# Autodesk Inventor assembly: Raspberry Pi 3
(part 2 of 2)
276. Raspberry Pi 3319_276
277. Raspberry Pi 3320_277
278. Raspberry Pi 3321_278
279. Raspberry Pi 3322_279
280. Raspberry Pi 3323_280
281. Raspberry Pi 3324_281
282. Raspberry Pi 3325_282
283. Raspberry Pi 3326_283
284. Raspberry Pi 3327_284
285. Raspberry Pi 3328_285
286. Raspberry Pi 3329_286
287. Raspberry Pi 3330_287
288. Raspberry Pi 3331_288
289. Raspberry Pi 3332_289
290. Raspberry Pi 3333_290
291. Raspberry Pi 3334_291
292. Raspberry Pi 3335_292
293. Raspberry Pi 3336_293
294. Raspberry Pi 3337_294
295. Raspberry Pi 3338_295
296. Raspberry Pi 3339_296
297. Raspberry Pi 3340_297
298. Raspberry Pi 3341_298
299. Raspberry Pi 3342_299
300. Raspberry Pi 3343_300
301. Raspberry Pi 3344_301
302. Raspberry Pi 3345_302
303. Raspberry Pi 3346_303
304. Raspberry Pi 3347_304
305. Raspberry Pi 3348_305
306. Raspberry Pi 3349_306
307. Raspberry Pi 3350_307
308. Raspberry Pi 3351_308
309. Raspberry Pi 3352_309
310. Raspberry Pi 3353_310
311. Raspberry Pi 3354_311
312. Raspberry Pi 327_312
313. Raspberry Pi 340_313
314. Raspberry Pi 344_314
315. Raspberry Pi 344_315
316. Raspberry Pi 340_316
317. Raspberry Pi 344_317
318. Raspberry Pi 340_318
319. Raspberry Pi 344_319
320. Raspberry Pi 340_320
321. Raspberry Pi 344_321
322. Raspberry Pi 340_322
323. Raspberry Pi 340_323
324. Raspberry Pi 344_324
325. Raspberry Pi 340_325
326. Raspberry Pi 344_326
327. Raspberry Pi 3357_327
328. Raspberry Pi 3355_328
329. Raspberry Pi 3356_329
330. Raspberry Pi 374_330
331. Raspberry Pi 3141_331
332. Raspberry Pi 374_332
333. Raspberry Pi 374_333
334. Raspberry Pi 374_334
335. Part2^Raspberry Pi 3_335
336. Raspberry Pi 3360_336
337. Part4^Raspberry Pi 3_337
338. Raspberry Pi 3159_338
339. Raspberry Pi 3158_339
340. Raspberry Pi 3160_340
341. Raspberry Pi 3162_341
342. Raspberry Pi 3161_342
343. Raspberry Pi 359_343
344. Raspberry Pi 3165_344
345. Raspberry Pi 353_345
346. Raspberry Pi 3164_346
347. Raspberry Pi 3163_347
348. Raspberry Pi 355_348
349. Raspberry Pi 3168_349
350. Raspberry Pi 3170_350
351. Raspberry Pi 3169_351
352. Raspberry Pi 3171_352
353. Raspberry Pi 3167_353
354. Raspberry Pi 3166_354
355. Raspberry Pi 353_355
356. Raspberry Pi 3165_356
357. Raspberry Pi 3163_357
358. Raspberry Pi 3164_358
359. Solder2_359
360. Solder2_360
361. Solder2_361
362. Solder2_362
363. Solder2_363
364. Solder2_364
365. Solder2_365
366. Solder2_366
367. Solder2_367
368. Solder2_368
369. Solder2_369
370. Raspberry Pi 3359_370
371. Solder2_371
372. Solder2_372
373. Solder2_373
374. Solder2_374
375. Solder2_375
376. Solder2_376
377. Solder2_377
378. Solder2_378
379. Solder2_379
380. Solder2_380
381. Solder2_381
382. Solder2_382
383. mf-msmf050-2_383
384. Solder2_384
385. Raspberry Pi 3163_smaller_385
386. Raspberry Pi 353_smaller_386
387. Raspberry Pi 3164_small_387
388. Raspberry Pi 3165_smaller_388
389. Raspberry Pi 3163_smaller_389
390. Raspberry Pi 353_smaller_390
391. Raspberry Pi 3164_small_391
392. Raspberry Pi 3165_smaller_392
393. Raspberry Pi 3163_smaller_393
394. Raspberry Pi 353_smaller_394
395. Raspberry Pi 3164_small_395
396. Raspberry Pi 3165_smaller_396
397. Raspberry Pi 3141_397
398. Raspberry Pi 3141_398
399. Raspberry Pi 3141_399
400. Raspberry Pi 3141_400
401. Raspberry Pi 3141_401
402. Raspberry Pi 3141_402
403. Raspberry Pi 3141_403
404. Raspberry Pi 3141_404
405. Raspberry Pi 3141_405
406. Raspberry Pi 3141_406
407. Raspberry Pi 3141_407
408. Raspberry Pi 3141_408
409. Raspberry Pi 3141_409
410. Raspberry Pi 3141_410
411. Raspberry Pi 3141_411
412. Raspberry Pi 3141_412
413. Raspberry Pi 3141_413
414. Raspberry Pi 3141_414
415. Raspberry Pi 3141_415
416. Raspberry Pi 3141_416
417. Raspberry Pi 3141_417
418. Raspberry Pi 3141_418
419. Raspberry Pi 3141_419
420. Raspberry Pi 3141_420
421. Raspberry Pi 3141_421
422. Raspberry Pi 3141_422
423. Raspberry Pi 3141_423
424. Raspberry Pi 3141_424
425. Raspberry Pi 3141_425
426. Raspberry Pi 3141_426
427. Raspberry Pi 3141_427
428. Raspberry Pi 3141_428
429. Raspberry Pi 3141_429
430. Raspberry Pi 3141_430
431. Raspberry Pi 3141_431
432. Raspberry Pi 3141_432
433. Raspberry Pi 3141_433
434. Raspberry Pi 3141_434
435. Raspberry Pi 3141_435
436. Raspberry Pi 3141_436
437. Raspberry Pi 3141_437
438. Raspberry Pi 3141_438
439. Raspberry Pi 3141_439
440. Raspberry Pi 3141_440
441. Raspberry Pi 3141_441
442. Raspberry Pi 3141_442
443. Raspberry Pi 3141_443
444. Raspberry Pi 3141_444
445. Raspberry Pi 3141_445
446. Raspberry Pi 3141_446
447. Raspberry Pi 3141_447
448. Raspberry Pi 3141_448
449. Raspberry Pi 3141_449
450. Raspberry Pi 3141_450
451. Raspberry Pi 3141_451
452. Raspberry Pi 3141_452
453. Raspberry Pi 3141_453
454. Raspberry Pi 3141_454
455. Raspberry Pi 374_455
456. Raspberry Pi 3141_456
457. Raspberry Pi 3141_457
458. Raspberry Pi 3141_458
459. Raspberry Pi 3141_459
460. Raspberry Pi 3141_460
461. Raspberry Pi 3141_461
462. Raspberry Pi 3141_462
463. Raspberry Pi 3141_463
464. Raspberry Pi 3141_464
465. Raspberry Pi 3141_465
466. Raspberry Pi 3141_466
467. Raspberry Pi 3141_467
468. Raspberry Pi 3141_468
469. Raspberry Pi 3141_469
470. Raspberry Pi 3141_470
471. Raspberry Pi 3141_471
472. Raspberry Pi 3141_472
473. Raspberry Pi 3141_473
474. Raspberry Pi 3141_474
475. Raspberry Pi 3141_475
476. Raspberry Pi 3141_476
477. Raspberry Pi 3141_477
478. Raspberry Pi 3141_478
479. Raspberry Pi 3141_479
480. Raspberry Pi 3141_480
481. Raspberry Pi 3141_481
482. Raspberry Pi 3141_482
483. Raspberry Pi 3141_smaller_483
484. Raspberry Pi 3141_smaller_484
485. Raspberry Pi 3141_smaller_485
486. Raspberry Pi 3141_smaller_486
487. Raspberry Pi 3141_smaller_487
488. Raspberry Pi 3141_smaller_488
489. Raspberry Pi 3141_smaller_489
490. Raspberry Pi 3141_smaller_490
491. Raspberry Pi 3141_smaller_491
492. Raspberry Pi 3141_smaller_492
493. Raspberry Pi 3141_smaller_493
494. Raspberry Pi 3141_smaller_494
495. Raspberry Pi 3141_smaller_495
496. Raspberry Pi 3141_smaller_496
497. Raspberry Pi 3141_smaller_497
498. Raspberry Pi 3141_smaller_498
499. Raspberry Pi 3141_smaller_499
500. Raspberry Pi 3141_smaller_500
501. Raspberry Pi 3141_smaller_501
502. Raspberry Pi 3141_smaller_502
503. Raspberry Pi 3141_smaller_503
504. Raspberry Pi 3141_smaller_504
505. Raspberry Pi 3141_smaller_505
506. Raspberry Pi 3141_smaller_506
507. Raspberry Pi 3141_smaller_507
508. Raspberry Pi 3281_508
509. Raspberry Pi 3280_509
510. Raspberry Pi 3282_510
511. Raspberry Pi 3285_511
512. Raspberry Pi 3283_512
513. Raspberry Pi 3284_513
514. Raspberry Pi 34_514
515. Raspberry Pi 3141_smaller_515
516. Raspberry Pi 3141_smaller_516
517. Raspberry Pi 3141_smaller_517
518. Raspberry Pi 3141_smaller_518
519. Raspberry Pi 3141_smaller_519
520. Raspberry Pi 3141_smaller_520
521. Raspberry Pi 3141_smaller_521
522. Raspberry Pi 3141_smaller_522
523. Raspberry Pi 3141_smaller_523
524. Raspberry Pi 3141_smaller_524
525. Raspberry Pi 3141_smaller_525
526. Raspberry Pi 3141_smaller_526
527. Raspberry Pi 3141_smaller_527
528. Raspberry Pi 3141_smaller_528
529. Raspberry Pi 3141_529
530. Raspberry Pi 345_530
531. Raspberry Pi 345_531
532. Raspberry Pi 345_532
533. Raspberry Pi 345_533
534. Raspberry Pi 3141_smaller_534
535. Solder2_535
536. Solder2_536
537. Solder2_537
538. Solder2_538
539. Solder2_539
540. Solder2_540
541. Solder2_541
542. Solder2_542
543. Solder2_543
544. Solder2_544
545. Solder2_545
546. Solder2_546
547. Solder2_547
548. Solder2_548
549. Solder2_549
550. Solder2_550
551. Solder2_551
552. Solder2_552
553. Solder2_553
554. Solder2_554
555. Solder2_555
556. Solder2_556
557. Solder2_557
558. Solder2_558
559. Solder2_559
560. Solder2_560
561. Solder2_561
562. Solder2_562
563. Solder2_563
564. Solder2_564
565. Solder2_565
566. Solder2_566
567. Solder2_567
568. Solder2_568
569. Solder2_569
570. Solder2_570
571. Solder2_571
572. Solder2_572
573. Solder2_573
574. Solder2_574
575. Solder2_575
576. Solder2_576
577. Solder2_577
578. Solder2_578
579. Solder2_579
580. Solder2_580
581. Solder2_581
582. Solder2_582
583. Solder2_583
584. Solder2_584
585. Solder2_585
586. Solder2_586
587. Solder2_587
588. Solder2_588
589. Solder2_589
590. Solder2_590
591. Solder2_591
592. Solder2_592
593. Solder2_593
594. raspberry_pi_B+_(microsd2)_594
595. Raspberry Pi 3242_595
596. Raspberry Pi 3242_596
597. Raspberry Pi 3242_597
598. Raspberry Pi 3242_598
599. Raspberry Pi 3242_599
600. Raspberry Pi 3242_600
601. Raspberry Pi 3242_601
602. Raspberry Pi 3242_602
603. Raspberry Pi 3242_603
604. Raspberry Pi 3242_604
605. Raspberry Pi 3242_605
606. Raspberry Pi 3242_606
607. Raspberry Pi 3242_607
608. Raspberry Pi 3242_608
609. Raspberry Pi 3242_609
610. Raspberry Pi 3242_610
611. Raspberry Pi 3242_611
612. Raspberry Pi 3242_612
613. Raspberry Pi 3242_613
614. Raspberry Pi 3266_614
615. Raspberry Pi 3266_615
616. Raspberry Pi 3266_616
617. Raspberry Pi 3266_617
618. Raspberry Pi 3266_618
619. Raspberry Pi 3266_619
620. Raspberry Pi 3266_620
621. Raspberry Pi 3266_621
622. Raspberry Pi 3266_622
623. Raspberry Pi 3266_623
624. Raspberry Pi 3266_624
625. Raspberry Pi 3266_625
626. Raspberry Pi 3266_626
627. Raspberry Pi 3266_627
628. Raspberry Pi 3266_628
629. Raspberry Pi 3266_629
630. Raspberry Pi 3266_630
631. Raspberry Pi 3266_631
632. Raspberry Pi 3266_632
633. raspberry_pi_B_(RJ45)_633
